# Autodesk Inventor assembly: box3
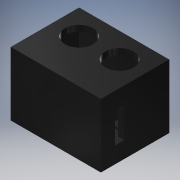
[picture p0: Inventor's stored thumbnail of the model, 180x180]
Saved by Autodesk Inventor 2019 (Build 230136000, 136)
## iProperties
Created: 2018-06-06
Part Number: box3
Document SubType Name: Assembly
Designer: stra92745
Author: stra92745
## Documents named in this file (7)
- C:\Users\stra92745\source\Workspaces\et-sys-dev\ET Internal Projects\SSTrolley\Dev\hardware\boxes\box3\box3.iam
- C:\Users\stra92745\source\Workspaces\et-sys-dev\ET Internal Projects\SSTrolley\Dev\hardware\boxes\box3\back.ipt
- C:\Users\stra92745\source\Workspaces\et-sys-dev\ET Internal Projects\SSTrolley\Dev\hardware\boxes\box3\bottom.ipt
- C:\Users\stra92745\source\Workspaces\et-sys-dev\ET Internal Projects\SSTrolley\Dev\hardware\boxes\box3\front.ipt
- C:\Users\stra92745\source\Workspaces\et-sys-dev\ET Internal Projects\SSTrolley\Dev\hardware\boxes\box3\left.ipt
- C:\Users\stra92745\source\Workspaces\et-sys-dev\ET Internal Projects\SSTrolley\Dev\hardware\boxes\box3\right.ipt
- C:\Users\stra92745\source\Workspaces\et-sys-dev\ET Internal Projects\SSTrolley\Dev\hardware\boxes\box3\top.ipt
## Components (6 placed, 6 different names)
1. back:1 — Mate:4, Mate:5, Mate:6, Mate:9, Mate:11, Flush:1, Mate:15, Mate:16
2. bottom:1 — Mate:1, Mate:2, Mate:3, Mate:4, Mate:5, Mate:6, Mate:7, Mate:8, Mate:10, Mate:12, Mate:13, Flush:2
3. front:1 — Mate:12, Mate:13, Flush:2, Mate:14
4. left:1 — Mate:7, Mate:8, Mate:9
5. right:1 — Mate:10, Mate:11, Flush:1
6. top:1 — Mate:14, Mate:15, Mate:16
## Relationships (18: Mate 16, Flush 2)
- Mate:1: bottom:1
- Mate:2: bottom:1
- Mate:3: bottom:1
- Mate:4: back:1 ↔ bottom:1
- Mate:5: back:1 ↔ bottom:1
- Mate:6: back:1 ↔ bottom:1
- Mate:7: bottom:1 ↔ left:1
- Mate:8: bottom:1 ↔ left:1
- Mate:9: back:1 ↔ left:1
- Mate:10: bottom:1 ↔ right:1
- Mate:11: back:1 ↔ right:1
- Flush:1: back:1 ↔ right:1
- Mate:12: bottom:1 ↔ front:1
- Mate:13: bottom:1 ↔ front:1
- Flush:2: bottom:1 ↔ front:1
- Mate:14: front:1 ↔ top:1
- Mate:15: back:1 ↔ top:1
- Mate:16: back:1 ↔ top:1
